# Autodesk Inventor assembly: Pneumatic Hub
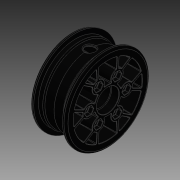
[picture p0: Inventor's stored thumbnail of the model, 180x180]
Saved by Autodesk Inventor 2014 SP1 (Build 180222100, 222)
## iProperties
Created: 2013-01-29
Part Number: Pneumatic Hub
Document SubType Name: Assembly
Designer: actoennies
Mass: 168.181 g
Surface Area: 833.094 cm^2
Volume: 149.04 cm^3
Density: 1.12843 g/cm^3
Author: actoennies
## Documents named in this file (3)
- C:\Users\Moses\Documents\Inventor\Rebuilds\Rebuild Sally\Pneumatic Hub.iam
- C:\Users\Moses\Documents\Inventor\Rebuilds\Rebuild Sally\#4x1.00, Plastic Thread Rolling Screw, Pan Head, Cross Recessed, Zinc Plated (Plastic Applications)_Faste.ipt
- C:\Users\Moses\Documents\Inventor\Rebuilds\Rebuild Sally\Hub.ipt
## Components (8 placed, 2 different names)
1. #4x1.00, Plastic Thread Rolling Screw, Pan Head, Cross Recessed, Zinc Plated (Plastic Applications)_Faste:1 — Insert:4
2. Hub:1 — Insert:2, Insert:3, Insert:5, Insert:7, Mate:2
3. #4x1.00, Plastic Thread Rolling Screw, Pan Head, Cross Recessed, Zinc Plated (Plastic Applications)_Faste:2 — Insert:1
4. #4x1.00, Plastic Thread Rolling Screw, Pan Head, Cross Recessed, Zinc Plated (Plastic Applications)_Faste:3 — Insert:5
5. #4x1.00, Plastic Thread Rolling Screw, Pan Head, Cross Recessed, Zinc Plated (Plastic Applications)_Faste:4 — Insert:6
6. #4x1.00, Plastic Thread Rolling Screw, Pan Head, Cross Recessed, Zinc Plated (Plastic Applications)_Faste:5 — Insert:3
7. #4x1.00, Plastic Thread Rolling Screw, Pan Head, Cross Recessed, Zinc Plated (Plastic Applications)_Faste:6 — Insert:2
8. Hub:2 — Insert:1, Insert:4, Insert:6, Insert:7, Mate:2
## Relationships (8: Insert 7, Mate 1)
- Insert:1: #4x1.00, Plastic Thread Rolling Screw, Pan Head, Cross Recessed, Zinc Plated (Plastic Applications)_Faste:2 ↔ Hub:2
- Insert:2: Hub:1 ↔ #4x1.00, Plastic Thread Rolling Screw, Pan Head, Cross Recessed, Zinc Plated (Plastic Applications)_Faste:6
- Insert:3: Hub:1 ↔ #4x1.00, Plastic Thread Rolling Screw, Pan Head, Cross Recessed, Zinc Plated (Plastic Applications)_Faste:5
- Insert:4: #4x1.00, Plastic Thread Rolling Screw, Pan Head, Cross Recessed, Zinc Plated (Plastic Applications)_Faste:1 ↔ Hub:2
- Insert:5: Hub:1 ↔ #4x1.00, Plastic Thread Rolling Screw, Pan Head, Cross Recessed, Zinc Plated (Plastic Applications)_Faste:3
- Insert:6: #4x1.00, Plastic Thread Rolling Screw, Pan Head, Cross Recessed, Zinc Plated (Plastic Applications)_Faste:4 ↔ Hub:2
- Insert:7: Hub:1 ↔ Hub:2
- Mate:2: Hub:1 ↔ Hub:2
